# Autodesk Inventor assembly: base
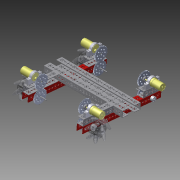
[picture p0: Inventor's stored thumbnail of the model, 180x180]
Saved by Autodesk Inventor 2015 (Build 190159000, 159)
## iProperties
Created: 2015-01-31
Part Number: base
Document SubType Name: Assembly
Designer: Bhaskar
Author: Bhaskar
## Documents named in this file (23)
- C:\Users\Bhaskar\Desktop\RoboCAD\base.iam
- C:\Users\Bhaskar\Desktop\Autodesk Workspace\FTC Parts\TETTRIX 416mm Aluminum Channel\Imported Components\Pitsco Education-739069\Assembly7.iam
- C:\Users\Bhaskar\Desktop\Autodesk Workspace\FTC Parts\TETTRIX 416mm Aluminum Channel\Imported Components\Pitsco Education-739069\Assembly12.iam
- C:\Users\Bhaskar\Desktop\RoboCAD\Imported Components\160mm Channel\Assembly13.iam
- C:\Users\Bhaskar\Desktop\RoboCAD\Imported Components\96mm Channel\Assembly14.iam
- C:\Users\Bhaskar\Desktop\RoboCAD\Imported Components\96mm Channel\Assembly15.iam
- C:\Users\Bhaskar\Desktop\RoboCAD\Imported Components\DC Motor Mount\Assembly16.iam
- C:\Users\Bhaskar\Desktop\RoboCAD\Imported Components\dc motor\Assembly17.iam
- C:\Users\Bhaskar\Desktop\RoboCAD\Imported Components\DC Motor Mount\Assembly19.iam
- C:\Users\Bhaskar\Desktop\RoboCAD\Imported Components\DC Motor Mount\Assembly20.iam
- C:\Users\Bhaskar\Desktop\RoboCAD\Imported Components\dc motor\Assembly21.iam
- C:\Users\Bhaskar\Desktop\RoboCAD\Imported Components\MotorShaftHub\Assembly22.iam
- C:\Users\Bhaskar\Desktop\RoboCAD\Imported Components\Medium Gear\Assembly24.iam
- C:\Users\Bhaskar\Desktop\RoboCAD\Imported Components\Axle\Assembly25.iam
- C:\Users\Bhaskar\Desktop\RoboCAD\Imported Components\BronzeBushing\Assembly26.iam
- C:\Users\Bhaskar\Desktop\RoboCAD\Imported Components\BronzeBushing\Assembly27.iam
- C:\Users\Bhaskar\Desktop\RoboCAD\Imported Components\Gear Hub Spacer\Assembly28.iam
- C:\Users\Bhaskar\Desktop\RoboCAD\Imported Components\Axle Hub\Assembly29.iam
- C:\Users\Bhaskar\Desktop\RoboCAD\leftMecanum.iam
- C:\Users\Bhaskar\Desktop\RoboCAD\Imported Components\BronzeBushing\Assembly31.iam
- C:\Users\Bhaskar\Desktop\RoboCAD\Imported Components\Axle Hub\Assembly33.iam
- C:\Users\Bhaskar\Desktop\RoboCAD\Imported Components\Axle\Assembly34.iam
- C:\Users\Bhaskar\Desktop\RoboCAD\Imported Components\Gear Hub Spacer\Assembly35.iam
## Components (49 placed, 22 different names)
1. Assembly12:1 [sub-assembly] — Insert:2, Insert:4
2. Assembly12:2 [sub-assembly] — Flush:1, Flush:2, Insert:4, Insert:5, Angle:2, Insert:7, Angle:4, Insert:31, Insert:32, Mate:26, Mate:28, Mate:31
3. Assembly12:3 [sub-assembly] — Insert:2, Insert:3, Angle:1, Flush:1, Flush:2, Insert:6, Angle:3, Insert:8, Angle:5, Insert:26, Insert:27, Insert:29, Insert:30
4. Assembly7:1 [sub-assembly] — Insert:3, Angle:1
5. Assembly13:1 [sub-assembly] — Insert:5, Angle:2, Insert:14, Angle:9
6. Assembly13:2 [sub-assembly] — Insert:6, Angle:3, Insert:13, Angle:8
7. Assembly14:1 [sub-assembly] — Insert:7, Angle:4, Insert:9, Angle:6
8. Assembly15:1 [sub-assembly] — Insert:8, Angle:5, Insert:10, Angle:7
9. Assembly16:1 [sub-assembly] — Insert:9, Angle:6, Insert:12
10. Assembly16:2 [sub-assembly] — Insert:10, Angle:7, Insert:11
11. Assembly17:1 [sub-assembly] — Insert:11, Insert:22
12. Assembly17:2 [sub-assembly] — Insert:12, Insert:24
13. Assembly19:1 [sub-assembly] — Insert:13, Angle:8, Insert:16
14. Assembly20:1 [sub-assembly] — Insert:14, Angle:9, Insert:15
15. Assembly21:1 [sub-assembly] — Insert:15, Insert:17
16. Assembly21:2 [sub-assembly] — Insert:16, Insert:19
17. Assembly22:1 [sub-assembly] — Insert:19, Insert:20
18. Assembly22:2 [sub-assembly] — Insert:17, Insert:21
19. Assembly24:1 [sub-assembly] — Insert:20, Rotation:3, Rotation:4
20. Assembly24:3 [sub-assembly] — Insert:21, Rotation:5
21. Assembly24:4 [sub-assembly] — Insert:23, Rotation:1, Rotation:2
22. Assembly22:3 [sub-assembly] — Insert:22, Insert:23
23. Assembly22:4 [sub-assembly] — Insert:24, Insert:25
24. Assembly24:5 [sub-assembly] — Insert:25, Flush:6
25. Assembly25:1 [sub-assembly] — Mate:1, Mate:2, Flush:3, Mate:3
26. Assembly26:1 [sub-assembly] — Insert:26, Mate:1, Mate:4
27. Assembly27:1 [sub-assembly] — Insert:27, Mate:5
28. Assembly28:1 [sub-assembly] — Mate:2, Flush:3, Mate:4, Mate:6, Mate:7
29. Assembly29:1 [sub-assembly] — Mate:3, Mate:5, Insert:28
30. Assembly24:6 [sub-assembly] — Insert:28, Rotation:1
31. leftMecanum:1 [sub-assembly] — Mate:6, Mate:7, Rotation:2
32. Assembly35:1 [sub-assembly] — Mate:9, Mate:10, Flush:4, Mate:16
33. Assembly34:1 [sub-assembly] — Mate:8, Mate:9, Flush:4, Mate:11, Mate:13, Mate:15
34. Assembly31:1 [sub-assembly] — Insert:30, Mate:8, Mate:12
35. Assembly31:2 [sub-assembly] — Insert:29, Mate:10
36. Assembly33:1 [sub-assembly] — Mate:11, Mate:12, Mate:14
37. Assembly24:8 [sub-assembly] — Mate:13, Mate:14, Rotation:3
38. leftMecanum:2 [sub-assembly] — Mate:15, Mate:16, Rotation:4
39. Assembly31:3 [sub-assembly] — Insert:31, Mate:21
40. Assembly31:4 [sub-assembly] — Insert:32, Mate:17, Mate:19
41. Assembly34:2 [sub-assembly] — Mate:17, Mate:18, Mate:20, Mate:22, Mate:24
42. Assembly35:2 [sub-assembly] — Mate:18, Mate:19, Mate:25
43. Assembly33:2 [sub-assembly] — Mate:20, Mate:21, Mate:23
44. Assembly24:9 [sub-assembly] — Mate:22, Mate:23, Rotation:5, Rotation:6
45. leftMecanum:3 [sub-assembly] — Mate:24, Mate:25, Rotation:6
46. Assembly34:3 [sub-assembly] — Mate:26, Mate:27, Flush:5, Mate:29, Mate:30
47. Assembly35:3 [sub-assembly] — Mate:27, Mate:28, Flush:5
48. Assembly24:10 [sub-assembly] — Mate:29, Flush:6
49. Assembly29:2 [sub-assembly] — Mate:30, Mate:31
## Relationships (82: Mate 31, Insert 30, Angle 9, Flush 6, RelateRotation 6)
- Insert:2: Assembly12:1 ↔ Assembly12:3
- Insert:3: Assembly12:3 ↔ Assembly7:1
- Angle:1 (0 deg): Assembly12:3 ↔ Assembly7:1
- Flush:1: Assembly12:2 ↔ Assembly12:3
- Flush:2: Assembly12:2 ↔ Assembly12:3
- Insert:4: Assembly12:1 ↔ Assembly12:2
- Insert:5: Assembly12:2 ↔ Assembly13:1
- Angle:2 (0 deg): Assembly12:2 ↔ Assembly13:1
- Insert:6: Assembly12:3 ↔ Assembly13:2
- Angle:3 (0 deg): Assembly12:3 ↔ Assembly13:2
- Insert:7: Assembly12:2 ↔ Assembly14:1
- Angle:4 (0 deg): Assembly12:2 ↔ Assembly14:1
- Insert:8: Assembly12:3 ↔ Assembly15:1
- Angle:5 (0 deg): Assembly12:3 ↔ Assembly15:1
- Insert:9: Assembly14:1 ↔ Assembly16:1
- Angle:6 (0 deg): Assembly14:1 ↔ Assembly16:1
- Insert:10: Assembly15:1 ↔ Assembly16:2
- Angle:7 (0 deg): Assembly15:1 ↔ Assembly16:2
- Insert:11: Assembly16:2 ↔ Assembly17:1
- Insert:12: Assembly16:1 ↔ Assembly17:2
- Insert:13: Assembly13:2 ↔ Assembly19:1
- Angle:8 (0 deg): Assembly13:2 ↔ Assembly19:1
- Insert:14: Assembly13:1 ↔ Assembly20:1
- Angle:9 (0 deg): Assembly13:1 ↔ Assembly20:1
- Insert:15: Assembly20:1 ↔ Assembly21:1
- Insert:16: Assembly19:1 ↔ Assembly21:2
- Insert:17: Assembly21:1 ↔ Assembly22:2
- Insert:19: Assembly21:2 ↔ Assembly22:1
- Insert:20: Assembly22:1 ↔ Assembly24:1
- Insert:21: Assembly22:2 ↔ Assembly24:3
- Insert:22: Assembly17:1 ↔ Assembly22:3
- Insert:23: Assembly24:4 ↔ Assembly22:3
- Insert:24: Assembly17:2 ↔ Assembly22:4
- Insert:25: Assembly22:4 ↔ Assembly24:5
- Insert:26: Assembly12:3 ↔ Assembly26:1
- Insert:27: Assembly12:3 ↔ Assembly27:1
- Mate:1: Assembly25:1 ↔ Assembly26:1
- Mate:2: Assembly25:1 ↔ Assembly28:1
- Flush:3: Assembly25:1 ↔ Assembly28:1
- Mate:3: Assembly25:1 ↔ Assembly29:1
- Mate:4: Assembly26:1 ↔ Assembly28:1
- Mate:5: Assembly27:1 ↔ Assembly29:1
- Insert:28: Assembly29:1 ↔ Assembly24:6
- Rotation:1 [RelateRotation] (1 ul): Assembly24:4 ↔ Assembly24:6
- Mate:6: Assembly28:1 ↔ leftMecanum:1
- Mate:7: Assembly28:1 ↔ leftMecanum:1
- Rotation:2 [RelateRotation] (1 ul): Assembly24:4 ↔ leftMecanum:1
- Insert:29: Assembly12:3 ↔ Assembly31:2
- Insert:30: Assembly12:3 ↔ Assembly31:1
- Mate:8: Assembly34:1 ↔ Assembly31:1
- Mate:9: Assembly35:1 ↔ Assembly34:1
- Mate:10: Assembly35:1 ↔ Assembly31:2
- Flush:4: Assembly35:1 ↔ Assembly34:1
- Mate:11: Assembly34:1 ↔ Assembly33:1
- Mate:12: Assembly31:1 ↔ Assembly33:1
- Mate:13: Assembly34:1 ↔ Assembly24:8
- Mate:14: Assembly33:1 ↔ Assembly24:8
- Rotation:3 [RelateRotation] (1 ul): Assembly24:1 ↔ Assembly24:8
- Mate:15: Assembly34:1 ↔ leftMecanum:2
- Mate:16: Assembly35:1 ↔ leftMecanum:2
- Rotation:4 [RelateRotation] (1 ul): Assembly24:1 ↔ leftMecanum:2
- Insert:31: Assembly12:2 ↔ Assembly31:3
- Insert:32: Assembly12:2 ↔ Assembly31:4
- Mate:17: Assembly31:4 ↔ Assembly34:2
- Mate:18: Assembly34:2 ↔ Assembly35:2
- Mate:19: Assembly31:4 ↔ Assembly35:2
- Mate:20: Assembly34:2 ↔ Assembly33:2
- Mate:21: Assembly31:3 ↔ Assembly33:2
- Mate:22: Assembly34:2 ↔ Assembly24:9
- Mate:23: Assembly33:2 ↔ Assembly24:9
- Rotation:5 [RelateRotation] (1 ul): Assembly24:3 ↔ Assembly24:9
- Mate:24: Assembly34:2 ↔ leftMecanum:3
- Mate:25: Assembly35:2 ↔ leftMecanum:3
- Rotation:6 [RelateRotation] (1 ul): Assembly24:9 ↔ leftMecanum:3
- Mate:26: Assembly12:2 ↔ Assembly34:3
- Mate:27: Assembly34:3 ↔ Assembly35:3
- Mate:28: Assembly12:2 ↔ Assembly35:3
- Flush:5: Assembly34:3 ↔ Assembly35:3
- Mate:29: Assembly34:3 ↔ Assembly24:10
- Flush:6: Assembly24:5 ↔ Assembly24:10
- Mate:30: Assembly34:3 ↔ Assembly29:2
- Mate:31: Assembly12:2 ↔ Assembly29:2
